# Autodesk Inventor assembly: Cajon
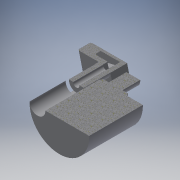
[picture p0: Inventor's stored thumbnail of the model, 180x180]
Saved by Autodesk Inventor 2019 (Build 230136000, 136)
## iProperties
Created: 2020-08-08
Part Number: Cajon
Document SubType Name: Assembly
Designer: Sergio
Author: Sergio
## Documents named in this file (4)
- C:\Users\Sergio\Documents\Innovandes\PROYECTO_GIT\EDITABLES\3D\VersionFinal\Anemometro\Ensambles\Cajon.iam
- C:\Users\Sergio\Documents\Innovandes\PROYECTO_GIT\EDITABLES\3D\VersionFinal\Anemometro\CajonInf.ipt
- C:\Users\Sergio\Documents\Innovandes\PROYECTO_GIT\EDITABLES\3D\VersionFinal\Anemometro\CajonSup.ipt
- C:\Users\Sergio\Documents\Innovandes\PROYECTO_GIT\EDITABLES\3D\VersionFinal\Anemometro\BaseEje.ipt
## Components (3 placed, 3 different names)
1. CajonInf:1 — Mate:1, Mate:2, Mate:3, Mate:4
2. CajonSup:1 — Mate:1, Mate:2, Mate:3
3. BaseEje:1 — Mate:4
## Relationships (4: Mate 4)
- Mate:1: CajonInf:1 ↔ CajonSup:1
- Mate:2: CajonInf:1 ↔ CajonSup:1
- Mate:3: CajonInf:1 ↔ CajonSup:1
- Mate:4: CajonInf:1 ↔ BaseEje:1
